# Autodesk Inventor assembly: Wheel
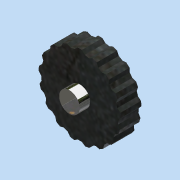
[picture p0: Inventor's stored thumbnail of the model, 180x180]
Saved by Autodesk Inventor 2015 (Build 190159000, 159)
## iProperties
Created: 2015-11-12
Part Number: Wheel
Document SubType Name: Assembly
Designer: Raphael
Author: Raphael
## Documents named in this file (3)
- \\psf\Home\Documents\electric-skateboard\Remote\CAD\Wheel.iam
- \\psf\Home\Documents\electric-skateboard\Remote\CAD\Wheel.ipt
- \\psf\Home\Documents\electric-skateboard\Remote\CAD\MagnetShaft.ipt
## Components (2 placed, 2 different names)
1. Wheel:1 — Mate:1
2. MagnetShaft:1 — Mate:1, Mate:2
## Relationships (2: Mate 2)
- Mate:1: Wheel:1 ↔ MagnetShaft:1
- Mate:2: MagnetShaft:1
